# Autodesk Inventor assembly: EnsamblajeMoto
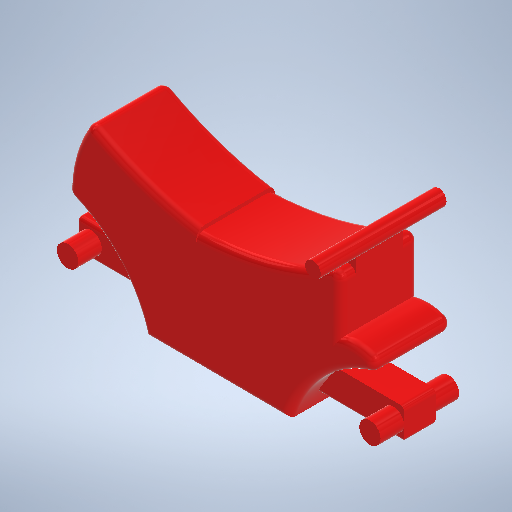
[picture p0: Inventor's stored thumbnail of the model, 512x512]
Saved by Autodesk Inventor 2025.1 (Build 291241000, 241)
## iProperties
Created: 2025-01-19
Part Number: EnsamblajeMoto
Document SubType Name: Assembly
Designer: usuario
Author: usuario
## Documents named in this file (3)
- C:\Users\yovan\Desktop\APM\ausol-apm.github.io\project\Design and simulation\Inventor\Modelado juguetes\Cad Juguetes\Moto\EnsamblajeMoto.iam
- C:\Users\yovan\Desktop\APM\ausol-apm.github.io\project\Design and simulation\Inventor\Modelado juguetes\Cad Juguetes\Moto\PiezaParteAtrasMoto.ipt
- C:\Users\yovan\Desktop\APM\ausol-apm.github.io\project\Design and simulation\Inventor\Modelado juguetes\Cad Juguetes\Moto\PiezaParteDelanteraMoto.ipt
## Components (2 placed, 2 different names)
1. PiezaParteAtrasMoto:1 — Mate:1, Flush:1, Flush:2
2. PiezaParteDelanteraMoto:1 — Mate:1, Flush:1, Flush:2
## Relationships (3: Flush 2, Mate 1)
- Mate:1: PiezaParteAtrasMoto:1 ↔ PiezaParteDelanteraMoto:1
- Flush:1: PiezaParteAtrasMoto:1 ↔ PiezaParteDelanteraMoto:1
- Flush:2: PiezaParteAtrasMoto:1 ↔ PiezaParteDelanteraMoto:1
